# Autodesk Inventor assembly: подшипник
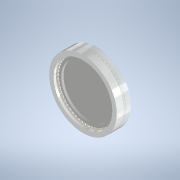
[picture p0: Inventor's stored thumbnail of the model, 180x180]
Saved by Autodesk Inventor 2020.1 (Build 241239000, 239)
## iProperties
Created: 2022-04-01
Part Number: подшипник
Document SubType Name: Assembly
Designer: User
Author: User
## Documents named in this file (3)
- D:\GitHub\TANK\3D-turret\подшипник.iam
- D:\GitHub\TANK\3D-turret\подшипник внешнее кольцо с шариками.iam
- D:\GitHub\TANK\3D-turret\внутреннее кольцо подшипника.ipt
## Components (3 placed, 2 different names)
1. подшипник внешнее кольцо с шариками:1 [sub-assembly] — Жесткий:1
2. подшипник внешнее кольцо с шариками:2 [sub-assembly] — Жесткий:1, Вставка:1
3. внутреннее кольцо подшипника:1 — Вставка:1
## Relationships (2: WeldJoint 1, Insert 1)
- Жесткий:1 [WeldJoint]: подшипник внешнее кольцо с шариками:1 ↔ подшипник внешнее кольцо с шариками:2
- Вставка:1 [Insert] (-15 mm): подшипник внешнее кольцо с шариками:2 ↔ внутреннее кольцо подшипника:1
